# Autodesk Inventor assembly: Ushape_all
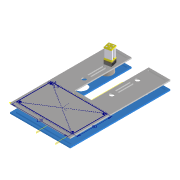
[picture p0: Inventor's stored thumbnail of the model, 180x180]
Saved by Autodesk Inventor 2020 (Build 240168000, 168)
## iProperties
Created: 2021-05-13
Part Number: Ushape_all
Document SubType Name: Assembly
Designer: Hsu Daniel
Author: Hsu Daniel
## Documents named in this file (5)
- D:\Daniel\NTU\makeNTU2021\大改\Ushape_all.iam
- D:\Daniel\NTU\makeNTU2021\大改\Ushape_bottom.ipt
- D:\Daniel\NTU\makeNTU2021\大改\Ushape_top.ipt
- D:\Daniel\NTU\makeNTU2021\大改\Stepper 28BYJ48.ipt
- D:\Daniel\NTU\makeNTU2021\大改\motor_connect.iam
## Components (4 placed, 4 different names)
1. Ushape_bottom:1 — Flush:1, Flush:2, Cylindrical:1, Flush:3
2. Ushape_top:1 — Flush:1, Flush:2, Insert:1
3. Stepper 28BYJ48:1 — Cylindrical:1, Insert:1, Flush:3, Mate:2, Cylindrical:2
4. motor_connect:1 [sub-assembly] — Mate:2, Cylindrical:2
## Relationships (7: Flush 3, CylindricalJoint 2, Insert 1, Mate 1)
- Flush:1: Ushape_bottom:1 ↔ Ushape_top:1
- Flush:2: Ushape_bottom:1 ↔ Ushape_top:1
- Cylindrical:1: Ushape_bottom:1 ↔ Stepper 28BYJ48:1
- Insert:1: Ushape_top:1 ↔ Stepper 28BYJ48:1
- Flush:3: Ushape_bottom:1 ↔ Stepper 28BYJ48:1
- Mate:2: Stepper 28BYJ48:1 ↔ motor_connect:1
- Cylindrical:2: Stepper 28BYJ48:1 ↔ motor_connect:1
